# Autodesk Inventor assembly: YAxisIdlerRight
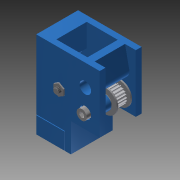
[picture p0: Inventor's stored thumbnail of the model, 180x180]
Saved by Autodesk Inventor 2015 SP1 (Build 190203100, 203)
## iProperties
Created: 2014-08-16
Part Number: YAxisIdlerRight
Document SubType Name: Assembly
Designer: Jack
Mass: 56.7089 g
Surface Area: 262.758 cm^2
Volume: 36.5041 cm^3
Density: 1.55349 g/cm^3
Author: Jack
Title: Y Idler Right
## Documents named in this file (11)
- C:\Users\Jack\ownCloud\Projects\CrossBot\InventorModel\YAxis\YAxisIdlerRight.iam
- C:\Users\Jack\ownCloud\Projects\CrossBot\InventorModel\YAxis\YAxisIdler\YIdlerCapRight.ipt
- C:\Users\Jack\ownCloud\Projects\CrossBot\InventorModel\Hardware\Bolts\SHCS\SHCS4\SHCS4x30.ipt
- C:\Users\Jack\ownCloud\Projects\CrossBot\InventorModel\Hardware\Nuts\Nut4.ipt
- C:\Users\Jack\ownCloud\Projects\CrossBot\InventorModel\Hardware\Bolts\SHCS\SHCS4\SHCS4x15.ipt
- C:\Users\Jack\ownCloud\Projects\CrossBot\InventorModel\Hardware\Wahsers\M4Washer.ipt
- C:\Users\Jack\ownCloud\Projects\CrossBot\InventorModel\Hardware\Belt\GT2Idler.iam
- C:\Users\Jack\ownCloud\Projects\CrossBot\InventorModel\YAxis\YAxisBeltIdlerSpacer.ipt
- C:\Users\Jack\ownCloud\Projects\CrossBot\InventorModel\Hardware\Bolts\FHS\FHS4\FHS4x8.ipt
- C:\Users\Jack\ownCloud\Projects\CrossBot\InventorModel\Hardware\Bolts\SHCS\SHCS4\SHCS4x8.ipt
- C:\Users\Jack\ownCloud\Projects\CrossBot\InventorModel\YAxis\YAxisIdler\YIdlerBlockRight.ipt
## Components (21 placed, 10 different names)
1. YIdlerCapRight:1 — Mate:18, Mate:15, Mate:17, Mate:16, Mate:77
2. SHCS4x30:1 — Mate:11, Mate:36, Mate:54, Mate:61, Mate:64, Mate:68, Mate:69
3. SHCS4x30:2 — Mate:13, Mate:35, Mate:50, Mate:58, Mate:59, Mate:66, Mate:67
4. Nut4:1 — Mate:11, Mate:74, Angle:1
5. Nut4:2 — Mate:13, Mate:73, Angle:2
6. SHCS4x15:1 — Mate:18, Mate:15, Mate:19, Mate:75
7. SHCS4x15:2 — Mate:17, Mate:16, Mate:20, Mate:76
8. Nut4:3 — Mate:19, Mate:62
9. Nut4:4 — Mate:20, Mate:63
10. M4Washer:1 — Mate:51, Mate:58, Mate:81
11. M4Washer:2 — Mate:35, Mate:53, Mate:60
12. M4Washer:3 — Mate:36, Mate:55, Mate:65
13. M4Washer:4 — Mate:56, Mate:64, Mate:80
14. GT2Idler:1 [sub-assembly] — Mate:50, Mate:51, Mate:53
15. GT2Idler:2 [sub-assembly] — Mate:54, Mate:55, Mate:56
16. YAxisBeltIdlerSpacer:1 — Mate:59, Mate:60
17. YAxisBeltIdlerSpacer:2 — Mate:61, Mate:65
18. FHS4x8:1 — Mate:78, Flush:2
19. SHCS4x8:1 — Mate:71, Mate:72
20. FHS4x8:2 — Mate:79, Flush:1
21. YIdlerBlockRight:1 — Mate:62, Mate:63, Mate:66, Mate:67, Mate:68, Mate:69, Mate:71, Mate:72, Mate:73, Mate:74, Angle:1, Angle:2, Mate:75, Mate:76, Mate:77, Mate:78, Mate:79, Flush:1, Flush:2, Mate:80, Mate:81
## Relationships (43: Mate 39, Angle 2, Flush 2)
- Mate:11: SHCS4x30:1 ↔ Nut4:1
- Mate:13: SHCS4x30:2 ↔ Nut4:2
- Mate:18: YIdlerCapRight:1 ↔ SHCS4x15:1
- Mate:15: YIdlerCapRight:1 ↔ SHCS4x15:1
- Mate:17: YIdlerCapRight:1 ↔ SHCS4x15:2
- Mate:16: YIdlerCapRight:1 ↔ SHCS4x15:2
- Mate:19: SHCS4x15:1 ↔ Nut4:3
- Mate:20: SHCS4x15:2 ↔ Nut4:4
- Mate:35: SHCS4x30:2 ↔ M4Washer:2
- Mate:36: SHCS4x30:1 ↔ M4Washer:3
- Mate:50: SHCS4x30:2 ↔ GT2Idler:1
- Mate:51: M4Washer:1 ↔ GT2Idler:1
- Mate:53: M4Washer:2 ↔ GT2Idler:1
- Mate:54: SHCS4x30:1 ↔ GT2Idler:2
- Mate:55: M4Washer:3 ↔ GT2Idler:2
- Mate:56: M4Washer:4 ↔ GT2Idler:2
- Mate:58: SHCS4x30:2 ↔ M4Washer:1
- Mate:59: SHCS4x30:2 ↔ YAxisBeltIdlerSpacer:1
- Mate:60: M4Washer:2 ↔ YAxisBeltIdlerSpacer:1
- Mate:61: SHCS4x30:1 ↔ YAxisBeltIdlerSpacer:2
- Mate:62: Nut4:3 ↔ YIdlerBlockRight:1
- Mate:63: Nut4:4 ↔ YIdlerBlockRight:1
- Mate:64: SHCS4x30:1 ↔ M4Washer:4
- Mate:65: M4Washer:3 ↔ YAxisBeltIdlerSpacer:2
- Mate:66: SHCS4x30:2 ↔ YIdlerBlockRight:1
- Mate:67: SHCS4x30:2 ↔ YIdlerBlockRight:1
- Mate:68: SHCS4x30:1 ↔ YIdlerBlockRight:1
- Mate:69: SHCS4x30:1 ↔ YIdlerBlockRight:1
- Mate:71: SHCS4x8:1 ↔ YIdlerBlockRight:1
- Mate:72: SHCS4x8:1 ↔ YIdlerBlockRight:1
- Mate:73: Nut4:2 ↔ YIdlerBlockRight:1
- Mate:74: Nut4:1 ↔ YIdlerBlockRight:1
- Angle:1 (0 deg): Nut4:1 ↔ YIdlerBlockRight:1
- Angle:2 (0 deg): Nut4:2 ↔ YIdlerBlockRight:1
- Mate:75: SHCS4x15:1 ↔ YIdlerBlockRight:1
- Mate:76: SHCS4x15:2 ↔ YIdlerBlockRight:1
- Mate:77: YIdlerCapRight:1 ↔ YIdlerBlockRight:1
- Mate:78: FHS4x8:1 ↔ YIdlerBlockRight:1
- Mate:79: FHS4x8:2 ↔ YIdlerBlockRight:1
- Flush:1: FHS4x8:2 ↔ YIdlerBlockRight:1
- Flush:2: FHS4x8:1 ↔ YIdlerBlockRight:1
- Mate:80: M4Washer:4 ↔ YIdlerBlockRight:1
- Mate:81: M4Washer:1 ↔ YIdlerBlockRight:1
